# Autodesk Inventor assembly: 3D_Drucker_v01
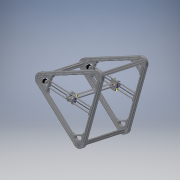
[picture p0: Inventor's stored thumbnail of the model, 180x180]
Saved by Autodesk Inventor 2019 (Build 230136000, 136)
## iProperties
Created: 2018-08-19
Part Number: 3D_Drucker_v01
Document SubType Name: Assembly
Designer: Julia
Author: Julia
## Documents named in this file (5)
- C:\Users\Julia\Documents\Inventor\3D_Drucker_v01\3D_Drucker_v01.iam
- C:\Users\Julia\Documents\Inventor\3D_Drucker_v01\Rahmen.iam
- C:\Users\Julia\Documents\Inventor\3D_Drucker_v01\Y_Führung.iam
- C:\Users\Julia\Documents\Inventor\M1173041- NEMA 17.ipt
- C:\Users\Julia\Documents\Inventor\3D_Drucker_v01\X_Führung.iam
## Components (6 placed, 4 different names)
1. Rahmen:1 [sub-assembly] — Mate:1, Mate:2, Mate:3, Mate:4, Mate:5, Mate:6, Mate:7, Mate:8, Mate:9, Mate:10, Mate:11, Mate:12
2. Y_Führung:1 [sub-assembly] — Mate:3, Mate:4, Mate:5, Mate:13, Mate:14
3. Y_Führung:2 [sub-assembly] — Mate:1, Mate:2, Mate:6
4. M1173041- NEMA 17:1 — Mate:7, Mate:8, Mate:9
5. M1173041- NEMA 17:2 — Mate:10, Mate:11, Mate:12
6. X_Führung:1 [sub-assembly] — Mate:13, Mate:14
## Relationships (14: Mate 14)
- Mate:1: Rahmen:1 ↔ Y_Führung:2
- Mate:2: Rahmen:1 ↔ Y_Führung:2
- Mate:3: Rahmen:1 ↔ Y_Führung:1
- Mate:4: Rahmen:1 ↔ Y_Führung:1
- Mate:5: Rahmen:1 ↔ Y_Führung:1
- Mate:6: Rahmen:1 ↔ Y_Führung:2
- Mate:7: Rahmen:1 ↔ M1173041- NEMA 17:1
- Mate:8: Rahmen:1 ↔ M1173041- NEMA 17:1
- Mate:9: Rahmen:1 ↔ M1173041- NEMA 17:1
- Mate:10: Rahmen:1 ↔ M1173041- NEMA 17:2
- Mate:11: Rahmen:1 ↔ M1173041- NEMA 17:2
- Mate:12: Rahmen:1 ↔ M1173041- NEMA 17:2
- Mate:13: Y_Führung:1 ↔ X_Führung:1
- Mate:14: Y_Führung:1 ↔ X_Führung:1
